# Autodesk Inventor assembly: pen_holder[_assembly
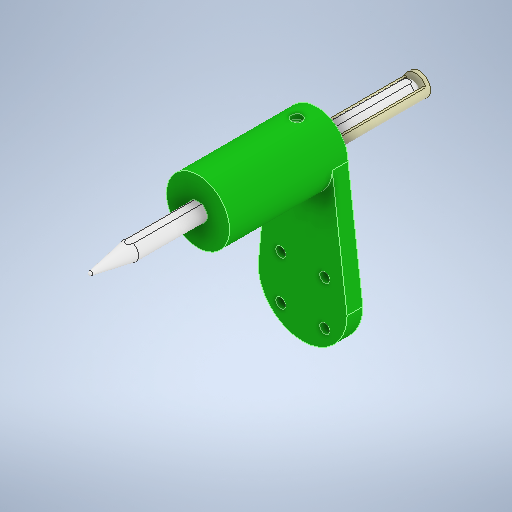
[picture p0: Inventor's stored thumbnail of the model, 512x512]
Saved by Autodesk Inventor 2025.1 (Build 291241000, 241)
## iProperties
Created: 2024-08-25
Part Number: pen_holder[_assembly
Document SubType Name: Assembly
Designer: pedro
Author: pedro
## Documents named in this file (4)
- C:\Users\pedro\OneDrive\Documentos\Inventor\prototipagem-3d-projeto\pen_holder_assembly.iam
- C:\Users\pedro\OneDrive\Documentos\Inventor\prototipagem-3d-projeto\pen_holder_2.ipt
- C:\Users\pedro\OneDrive\Documentos\Inventor\prototipagem-3d-projeto\stylus_pen_2.ipt
- C:\Users\pedro\OneDrive\Documentos\Inventor\prototipagem-3d-projeto\pen_limiter.ipt
## Components (3 placed, 3 different names)
1. pen_holder_2:1 — Mate:1, Mate:2, Mate:3
2. stylus_pen_2:1 — Mate:1
3. pen_limiter:1 — Mate:2, Mate:3
## Relationships (3: Mate 3)
- Mate:1: pen_holder_2:1 ↔ stylus_pen_2:1
- Mate:2: pen_holder_2:1 ↔ pen_limiter:1
- Mate:3: pen_holder_2:1 ↔ pen_limiter:1
